# Autodesk Inventor assembly: motor housing
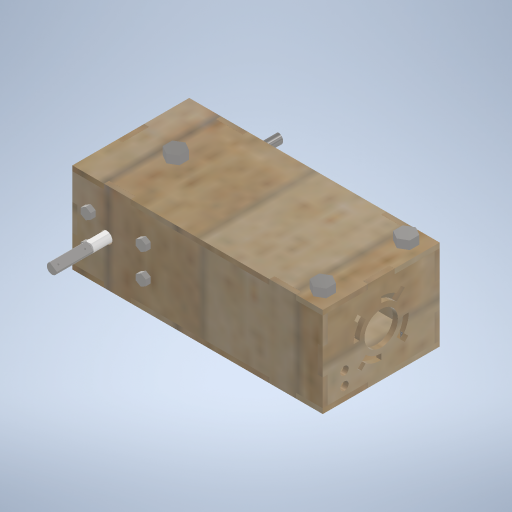
[picture p0: Inventor's stored thumbnail of the model, 512x512]
Saved by Autodesk Inventor 2023 (Build 270158000, 158)
## iProperties
Created: 2023-06-06
Part Number: motor housing
Document SubType Name: Assembly
Designer: Ronan
Author: Ronan
## Documents named in this file (10)
- D:\Libraries\Documents\2023-FYP\Inventor\motor housing.iam
- D:\Libraries\Documents\2023-FYP\Inventor\JGY-37012V JGY370-D7 DC Gearmotor.iam
- D:\Libraries\Documents\2023-FYP\Inventor\side plate.ipt
- D:\Libraries\Documents\2023-FYP\Inventor\m3 bolt.ipt
- D:\Libraries\Documents\2023-FYP\Inventor\bottom plate.ipt
- D:\Libraries\Documents\2023-FYP\Inventor\front plate.ipt
- D:\Libraries\Documents\2023-FYP\Inventor\back plate.ipt
- D:\Libraries\Documents\2023-FYP\Inventor\centre shaft.ipt
- D:\Libraries\Documents\2023-FYP\Inventor\m5-bolt-long.ipt
- D:\Libraries\Documents\2023-FYP\Inventor\M5-nut-4mm.ipt
## Components (24 placed, 9 different names)
1. JGY-37012V JGY370-D7 DC Gearmotor:1 [sub-assembly] — Cylindrical:1, Cylindrical:2, Mate:1, Mate:36, Mate:37, Rotation:2
2. side plate:1 — Cylindrical:1, Cylindrical:2, Mate:1, Mate:2, Mate:3, Mate:4, Mate:5, Mate:6, Mate:7, Mate:8, Mate:9, Mate:10, Mate:11, Mate:12, Mate:26, Mate:27, Mate:28, Mate:34
3. m3 bolt:1 — Mate:2, Mate:7
4. m3 bolt:2 — Mate:4, Mate:9
5. m3 bolt:3 — Mate:3, Mate:6
6. m3 bolt:4 — Mate:5, Mate:8
7. bottom plate:1 — Mate:10, Mate:11, Mate:12, Mate:13, Mate:23, Mate:24, Mate:25, Mate:47
8. JGY-37012V JGY370-D7 DC Gearmotor:2 [sub-assembly] — Mate:38, Mate:39, Rotation:1
9. side plate:3 — Mate:23, Mate:24, Mate:25, Mate:30, Mate:33
10. m3 bolt:5
11. m3 bolt:6
12. m3 bolt:7
13. m3 bolt:8
14. bottom plate:2 — Mate:26, Mate:27, Mate:28, Mate:29, Mate:31, Mate:32, Mate:40, Mate:41, Mate:42, Mate:43
15. front plate:1 — Mate:29, Mate:30, Mate:31, Mate:35
16. back plate:1 — Mate:32, Mate:33, Mate:34
17. Shaft:1 — Mate:36, Mate:37, Rotation:2
18. Shaft:2 — Mate:38, Mate:39, Rotation:1
19. m5-bolt-long:1 — Mate:41, Flush:2, Mate:44
20. m5-bolt-long:2 — Mate:40, Mate:43, Flush:1, Flush:2, Mate:45
21. m5-bolt-long:3 — Mate:42, Flush:1, Mate:46
22. M5-nut-4mm:1 — Mate:44, Flush:3
23. M5-nut-4mm:2 — Mate:45, Mate:47, Flush:3, Flush:4
24. M5-nut-4mm:3 — Mate:46, Flush:4
## Relationships (57: Mate 47, CylindricalJoint 4, Flush 4, RelateRotation 2)
- Cylindrical:1: JGY-37012V JGY370-D7 DC Gearmotor:1 ↔ side plate:1
- Cylindrical:2: JGY-37012V JGY370-D7 DC Gearmotor:1 ↔ side plate:1
- Mate:1: JGY-37012V JGY370-D7 DC Gearmotor:1 ↔ side plate:1
- Mate:2: side plate:1 ↔ m3 bolt:1
- Mate:3: side plate:1 ↔ m3 bolt:3
- Mate:4: side plate:1 ↔ m3 bolt:2
- Mate:5: side plate:1 ↔ m3 bolt:4
- Mate:6: side plate:1 ↔ m3 bolt:3
- Mate:7: side plate:1 ↔ m3 bolt:1
- Mate:8: side plate:1 ↔ m3 bolt:4
- Mate:9: side plate:1 ↔ m3 bolt:2
- Mate:10: side plate:1 ↔ bottom plate:1
- Mate:11: side plate:1 ↔ bottom plate:1
- Mate:12: side plate:1 ↔ bottom plate:1
- Mate:13: bottom plate:1
- [CylindricalJoint]: JGY-37012V JGY370-D7 DC Gearmotor:2 ↔ side plate:3
- [CylindricalJoint]: JGY-37012V JGY370-D7 DC Gearmotor:2 ↔ side plate:3
- [Mate]: JGY-37012V JGY370-D7 DC Gearmotor:2 ↔ side plate:3
- [Mate]: side plate:3 ↔ m3 bolt:5
- [Mate]: side plate:3 ↔ m3 bolt:7
- [Mate]: side plate:3 ↔ m3 bolt:6
- [Mate]: side plate:3 ↔ m3 bolt:8
- [Mate]: side plate:3 ↔ m3 bolt:7
- [Mate]: side plate:3 ↔ m3 bolt:5
- [Mate]: side plate:3 ↔ m3 bolt:8
- [Mate]: side plate:3 ↔ m3 bolt:6
- Mate:23: bottom plate:1 ↔ side plate:3
- Mate:24: bottom plate:1 ↔ side plate:3
- Mate:25: bottom plate:1 ↔ side plate:3
- Mate:26: side plate:1 ↔ bottom plate:2
- Mate:27: side plate:1 ↔ bottom plate:2
- Mate:28: side plate:1 ↔ bottom plate:2
- Mate:29: bottom plate:2 ↔ front plate:1
- Mate:30: side plate:3 ↔ front plate:1
- Mate:31: bottom plate:2 ↔ front plate:1
- Mate:32: bottom plate:2 ↔ back plate:1
- Mate:33: side plate:3 ↔ back plate:1
- Mate:34: side plate:1 ↔ back plate:1
- Mate:35: front plate:1
- Mate:36: JGY-37012V JGY370-D7 DC Gearmotor:1 ↔ Shaft:1
- Mate:37: JGY-37012V JGY370-D7 DC Gearmotor:1 ↔ Shaft:1
- Mate:38: JGY-37012V JGY370-D7 DC Gearmotor:2 ↔ Shaft:2
- Mate:39: JGY-37012V JGY370-D7 DC Gearmotor:2 ↔ Shaft:2
- Rotation:1 [RelateRotation] (-1 ul): JGY-37012V JGY370-D7 DC Gearmotor:2 ↔ Shaft:2
- Rotation:2 [RelateRotation] (-1 ul): JGY-37012V JGY370-D7 DC Gearmotor:1 ↔ Shaft:1
- Mate:40: bottom plate:2 ↔ m5-bolt-long:2
- Mate:41: bottom plate:2 ↔ m5-bolt-long:1
- Mate:42: bottom plate:2 ↔ m5-bolt-long:3
- Mate:43: bottom plate:2 ↔ m5-bolt-long:2
- Flush:1: m5-bolt-long:2 ↔ m5-bolt-long:3
- Flush:2: m5-bolt-long:1 ↔ m5-bolt-long:2
- Mate:44: m5-bolt-long:1 ↔ M5-nut-4mm:1
- Mate:45: m5-bolt-long:2 ↔ M5-nut-4mm:2
- Mate:46: m5-bolt-long:3 ↔ M5-nut-4mm:3
- Mate:47: bottom plate:1 ↔ M5-nut-4mm:2
- Flush:3: M5-nut-4mm:1 ↔ M5-nut-4mm:2
- Flush:4: M5-nut-4mm:2 ↔ M5-nut-4mm:3
## Named parameters: d20_d3 = 0.341768 deg, d21_d4 = -73.90041 mm, d22_d5 = 90 deg, d23_d6 = -60.15041 mm, d24_d7 = 0 mm, d25_d8 = 0 mm, d26_d9 = 0 mm, d27_d10 = 0 mm, d28_d11 = 0 mm, d29_d12 = 0 mm, d30_d13 = 0 mm, d31_d14 = 0 mm, d32_d15 = 0 mm
